# Autodesk Inventor assembly: Cerniera versione 3
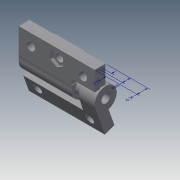
[picture p0: Inventor's stored thumbnail of the model, 180x180]
Saved by Autodesk Inventor 2019 (Build 230136000, 136)
## iProperties
Created: 2019-06-30
Part Number: Cerniera versione 3
Document SubType Name: Assembly
Designer: giacomo
Author: giacomo
## Documents named in this file (4)
- D:\Hobby\Inventor\Prove 3D printer\Cerniera\Versione 3\Cerniera versione 3.iam
- D:\Hobby\Inventor\Prove 3D printer\Cerniera\Versione 3\Cerniera 5.5.ipt
- D:\Hobby\Inventor\Prove 3D printer\Cerniera\Versione 3\Cerniera 5.ipt
- D:\Hobby\Inventor\Prove 3D printer\Cerniera\Versione 3\Cerniera 6.ipt
## Components (3 placed, 3 different names)
1. Cerniera 5.5:1 — Mate:1, Flush:2
2. Cerniera 5:1 — Mate:1, Mate:2
3. Cerniera 6:1 — Mate:2, Flush:2
## Relationships (3: Mate 2, Flush 1)
- Mate:1: Cerniera 5.5:1 ↔ Cerniera 5:1
- Mate:2: Cerniera 5:1 ↔ Cerniera 6:1
- Flush:2: Cerniera 5.5:1 ↔ Cerniera 6:1
